# Autodesk Inventor assembly: hela
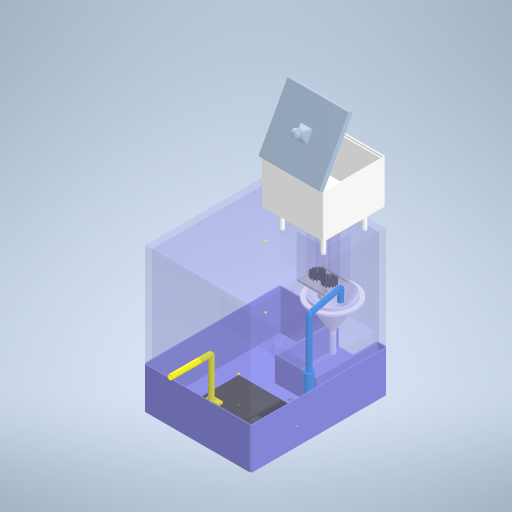
[picture p0: Inventor's stored thumbnail of the model, 512x512]
Saved by Autodesk Inventor 2023 (Build 270158000, 158)
## iProperties
Created: 2022-11-26
Part Number: hela
Document SubType Name: Assembly
Designer: abdul
Author: abdul
## Documents named in this file (9)
- C:\Users\abdul\OneDrive\Skrivbord\maskin design\cad\ASS\hela.iam
- C:\Users\abdul\OneDrive\Skrivbord\maskin design\cad\case.ipt
- C:\Users\abdul\OneDrive\Skrivbord\maskin design\cad\coffe container.ipt
- C:\Users\abdul\OneDrive\Skrivbord\maskin design\cad\coffee container lock.ipt
- C:\Users\abdul\OneDrive\Skrivbord\maskin design\cad\malare.ipt
- C:\Users\abdul\OneDrive\Skrivbord\maskin design\cad\tofilter.ipt
- C:\Users\abdul\OneDrive\Skrivbord\maskin design\cad\ASS\Filter.ipt
- C:\Users\abdul\OneDrive\Skrivbord\maskin design\cad\case_botten.ipt
- C:\Users\abdul\OneDrive\Skrivbord\maskin design\cad\ASS\System water kanjo.iam
## Components (9 placed, 8 different names)
1. case:1 — Mate:1, Mate:2, Mate:3, Mate:4, Mate:5, Flush:3, Flush:4, Flush:5, Mate:7, Mate:8, Tangent:1, Tangent:2, Mate:13, Mate:14, Mate:18, Mate:19, Flush:6, Mate:20
2. coffe container:1 — Mate:1, Mate:2, Mate:3, Mate:4, Mate:5, Mate:6, Flush:1
3. coffee container lock:1 — Mate:6, Flush:1
4. malare:1 — Flush:2, Flush:3, Flush:5, Mate:7
5. malare:2 — Flush:2, Flush:4, Mate:8
6. tofilter:1 — Mate:13, Mate:14
7. Filter:1 — Tangent:1, Tangent:2
8. case_botten:1 — Mate:15, Mate:16, Mate:17, Mate:18, Mate:19, Flush:6, Mate:20
9. System water kanjo:1 [sub-assembly] — Mate:15, Mate:16, Mate:17
## Relationships (24: Mate 16, Flush 6, Tangent 2)
- Mate:1: case:1 ↔ coffe container:1
- Mate:2: case:1 ↔ coffe container:1
- Mate:3: case:1 ↔ coffe container:1
- Mate:4: case:1 ↔ coffe container:1
- Mate:5: case:1 ↔ coffe container:1
- Mate:6: coffe container:1 ↔ coffee container lock:1
- Flush:1: coffe container:1 ↔ coffee container lock:1
- Flush:2: malare:1 ↔ malare:2
- Flush:3: case:1 ↔ malare:1
- Flush:4: case:1 ↔ malare:2
- Flush:5: case:1 ↔ malare:1
- Mate:7: case:1 ↔ malare:1
- Mate:8: case:1 ↔ malare:2
- Tangent:1: case:1 ↔ Filter:1
- Tangent:2: case:1 ↔ Filter:1
- Mate:13: case:1 ↔ tofilter:1
- Mate:14: case:1 ↔ tofilter:1
- Mate:15: case_botten:1 ↔ System water kanjo:1
- Mate:16: case_botten:1 ↔ System water kanjo:1
- Mate:17: case_botten:1 ↔ System water kanjo:1
- Mate:18: case:1 ↔ case_botten:1
- Mate:19: case:1 ↔ case_botten:1
- Flush:6: case:1 ↔ case_botten:1
- Mate:20: case:1 ↔ case_botten:1
